# Autodesk Inventor assembly: ASY Вал
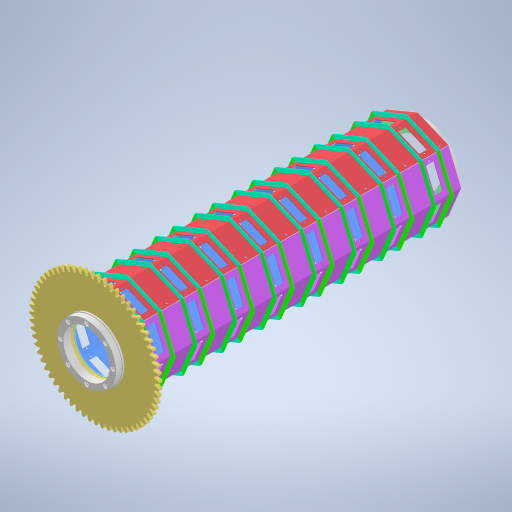
[picture p0: Inventor's stored thumbnail of the model, 512x512]
Saved by Autodesk Inventor 2024.2 (Build 282272000, 272)
## iProperties
Created: 2024-04-28
Part Number: ASY Вал
Document SubType Name: Assembly
Designer: pokla
Author: pokla
## Documents named in this file (13)
- C:\Users\admin\My Drive (bigstupidbeast@gmail.com)\Inventor\Disk Micro filter\ДМФ 06.05.24 21-33\ASY Вал.iam
- C:\Users\admin\My Drive (bigstupidbeast@gmail.com)\Inventor\Disk Micro filter\ДМФ 06.05.24 21-33\ДМС 101 Барабан торец.ipt
- C:\Users\admin\My Drive (bigstupidbeast@gmail.com)\Inventor\Disk Micro filter\ДМФ 06.05.24 21-33\ДМС 100 Барабан Лист №2.ipt
- C:\Users\admin\My Drive (bigstupidbeast@gmail.com)\Inventor\Disk Micro filter\ДМФ 06.05.24 21-33\ДМС 100 Барабан Лист №3.ipt
- C:\Users\admin\My Drive (bigstupidbeast@gmail.com)\Inventor\Disk Micro filter\ДМФ 06.05.24 21-33\ДМС 102 Опорное кольцо вала перед.ipt
- C:\Users\admin\My Drive (bigstupidbeast@gmail.com)\Inventor\Disk Micro filter\ДМФ 06.05.24 21-33\ДМС 103 Полка для крышки.ipt
- C:\Users\admin\My Drive (bigstupidbeast@gmail.com)\Inventor\Disk Micro filter\ДМФ 06.05.24 21-33\ДМС 000 размеры.ipt
- C:\Users\admin\My Drive (bigstupidbeast@gmail.com)\Inventor\Disk Micro filter\ДМФ 06.05.24 21-33\ДМС 105 Шестерня ведомая.ipt
- C:\Users\admin\My Drive (bigstupidbeast@gmail.com)\Inventor\Disk Micro filter\ДМФ 06.05.24 21-33\ДМС 104 Сектор кольца усилителя барабана_CPY.ipt
- C:\Users\admin\My Drive (bigstupidbeast@gmail.com)\Inventor\Disk Micro filter\ДМФ 06.05.24 21-33\ASY ДМФГиД 01010 крышка галка.iam
- C:\Users\admin\My Drive (bigstupidbeast@gmail.com)\Inventor\Disk Micro filter\ДМФ 06.05.24 21-33\ASY ДМФГиД 01011 Кассета.iam
- C:\Users\admin\My Drive (bigstupidbeast@gmail.com)\Inventor\Disk Micro filter\ДМФ 06.05.24 21-33\ДМС 103 Опорное кольцо вала хвост.ipt.ipt
- ДМС 103 Опорное кольцо вала хвост.ipt
## Components (123 placed, 11 different names)
1. ДМС 000 размеры:1
2. ДМС 101 Барабан торец:2 — Rotational:5, Mate:7, Rigid:15, Rigid:16, Mate:8, Flush:1, Flush:2, Mate:9, Flush:3, Flush:4, Mate:10, Flush:5, Flush:6
3. ДМС 101 Барабан торец:1 — Rotational:6
4. ДМС 100 Барабан Лист №2:1 — Rigid:15, Mate:12, Flush:7
5. ДМС 100 Барабан Лист №3:1 — Rigid:16, Mate:11
6. ДМС 102 Опорное кольцо вала перед:1 — Mate:1, Mate:2, Rotational:4, Mate:6, Rotational:5
7. ДМС 103 Полка для крышки:1 — Mate:9, Flush:3, Flush:4
8. ДМС 103 Полка для крышки:2 — Mate:8, Flush:1, Flush:2
9. ДМС 105 Шестерня ведомая:1 — Rotational:4, Mate:6
10. ASY ДМФГиД 01010 крышка галка:1 [sub-assembly] — Mate:10, Flush:5, Flush:6, Rigid:17
11. ДМС 103 Опорное кольцо вала хвост.ipt:1 — Rotational:6
12. ДМС 104 Сектор кольца усилителя барабана_CPY:4 — Rigid:10
13. ДМС 104 Сектор кольца усилителя барабана_CPY:1 — Rigid:8
14. ДМС 104 Сектор кольца усилителя барабана_CPY:5 — Rigid:10, Rigid:11, Rigid:14
15. ДМС 104 Сектор кольца усилителя барабана_CPY:2 — Rigid:8, Rigid:9, Rigid:14
16. ДМС 104 Сектор кольца усилителя барабана_CPY:3 — Rigid:9, Mate:12
17. ДМС 104 Сектор кольца усилителя барабана_CPY:6 — Rigid:11
18. ДМС 104 Сектор кольца усилителя барабана_CPY:7
19. ДМС 104 Сектор кольца усилителя барабана_CPY:8
20. ДМС 104 Сектор кольца усилителя барабана_CPY:21
21. ДМС 104 Сектор кольца усилителя барабана_CPY:28
22. ДМС 104 Сектор кольца усилителя барабана_CPY:35
23. ДМС 104 Сектор кольца усилителя барабана_CPY:42
24. ДМС 104 Сектор кольца усилителя барабана_CPY:9
25. ДМС 104 Сектор кольца усилителя барабана_CPY:10
26. ДМС 104 Сектор кольца усилителя барабана_CPY:22
27. ДМС 104 Сектор кольца усилителя барабана_CPY:29
28. ДМС 104 Сектор кольца усилителя барабана_CPY:36
29. ДМС 104 Сектор кольца усилителя барабана_CPY:43
30. ДМС 104 Сектор кольца усилителя барабана_CPY:11
31. ДМС 104 Сектор кольца усилителя барабана_CPY:12
32. ДМС 104 Сектор кольца усилителя барабана_CPY:23
33. ДМС 104 Сектор кольца усилителя барабана_CPY:30
34. ДМС 104 Сектор кольца усилителя барабана_CPY:37
35. ДМС 104 Сектор кольца усилителя барабана_CPY:44
36. ДМС 104 Сектор кольца усилителя барабана_CPY:13
37. ДМС 104 Сектор кольца усилителя барабана_CPY:14
38. ДМС 104 Сектор кольца усилителя барабана_CPY:24
39. ДМС 104 Сектор кольца усилителя барабана_CPY:31
40. ДМС 104 Сектор кольца усилителя барабана_CPY:38
41. ДМС 104 Сектор кольца усилителя барабана_CPY:45
42. ДМС 104 Сектор кольца усилителя барабана_CPY:15
43. ДМС 104 Сектор кольца усилителя барабана_CPY:16
44. ДМС 104 Сектор кольца усилителя барабана_CPY:25
45. ДМС 104 Сектор кольца усилителя барабана_CPY:32
46. ДМС 104 Сектор кольца усилителя барабана_CPY:39
47. ДМС 104 Сектор кольца усилителя барабана_CPY:46
48. ДМС 104 Сектор кольца усилителя барабана_CPY:17
49. ДМС 104 Сектор кольца усилителя барабана_CPY:18
50. ДМС 104 Сектор кольца усилителя барабана_CPY:26
51. ДМС 104 Сектор кольца усилителя барабана_CPY:33
52. ДМС 104 Сектор кольца усилителя барабана_CPY:40
53. ДМС 104 Сектор кольца усилителя барабана_CPY:47
54. ДМС 104 Сектор кольца усилителя барабана_CPY:19 — Mate:11
55. ДМС 104 Сектор кольца усилителя барабана_CPY:20
56. ДМС 104 Сектор кольца усилителя барабана_CPY:27
57. ДМС 104 Сектор кольца усилителя барабана_CPY:34
58. ДМС 104 Сектор кольца усилителя барабана_CPY:41
59. ДМС 104 Сектор кольца усилителя барабана_CPY:48 — Flush:7
60. ASY ДМФГиД 01011 Кассета:1 [sub-assembly] — Rigid:17
61. ASY ДМФГиД 01011 Кассета:2 [sub-assembly]
62. ASY ДМФГиД 01011 Кассета:3 [sub-assembly]
63. ASY ДМФГиД 01011 Кассета:4 [sub-assembly]
64. ASY ДМФГиД 01011 Кассета:5 [sub-assembly]
65. ASY ДМФГиД 01011 Кассета:6 [sub-assembly]
66. ASY ДМФГиД 01011 Кассета:7 [sub-assembly]
67. ASY ДМФГиД 01011 Кассета:8 [sub-assembly]
68. ASY ДМФГиД 01011 Кассета:9 [sub-assembly]
69. ASY ДМФГиД 01011 Кассета:10 [sub-assembly]
70. ASY ДМФГиД 01011 Кассета:11 [sub-assembly]
71. ASY ДМФГиД 01011 Кассета:12 [sub-assembly]
72. ASY ДМФГиД 01011 Кассета:13 [sub-assembly]
73. ASY ДМФГиД 01011 Кассета:14 [sub-assembly]
74. ASY ДМФГиД 01011 Кассета:15 [sub-assembly]
75. ASY ДМФГиД 01011 Кассета:16 [sub-assembly]
76. ASY ДМФГиД 01011 Кассета:17 [sub-assembly]
77. ASY ДМФГиД 01011 Кассета:18 [sub-assembly]
78. ASY ДМФГиД 01011 Кассета:19 [sub-assembly]
79. ASY ДМФГиД 01011 Кассета:20 [sub-assembly]
80. ASY ДМФГиД 01011 Кассета:21 [sub-assembly]
81. ASY ДМФГиД 01011 Кассета:22 [sub-assembly]
82. ASY ДМФГиД 01011 Кассета:23 [sub-assembly]
83. ASY ДМФГиД 01011 Кассета:24 [sub-assembly]
84. ASY ДМФГиД 01011 Кассета:25 [sub-assembly]
85. ASY ДМФГиД 01011 Кассета:26 [sub-assembly]
86. ASY ДМФГиД 01011 Кассета:27 [sub-assembly]
87. ASY ДМФГиД 01011 Кассета:28 [sub-assembly]
88. ASY ДМФГиД 01011 Кассета:29 [sub-assembly]
89. ASY ДМФГиД 01011 Кассета:30 [sub-assembly]
90. ASY ДМФГиД 01011 Кассета:31 [sub-assembly]
91. ASY ДМФГиД 01011 Кассета:32 [sub-assembly]
92. ASY ДМФГиД 01011 Кассета:33 [sub-assembly]
93. ASY ДМФГиД 01011 Кассета:34 [sub-assembly]
94. ASY ДМФГиД 01011 Кассета:35 [sub-assembly]
95. ASY ДМФГиД 01011 Кассета:36 [sub-assembly]
96. ASY ДМФГиД 01011 Кассета:37 [sub-assembly]
97. ASY ДМФГиД 01011 Кассета:38 [sub-assembly]
98. ASY ДМФГиД 01011 Кассета:39 [sub-assembly]
99. ASY ДМФГиД 01011 Кассета:40 [sub-assembly]
100. ASY ДМФГиД 01011 Кассета:41 [sub-assembly]
101. ASY ДМФГиД 01011 Кассета:42 [sub-assembly]
102. ASY ДМФГиД 01011 Кассета:43 [sub-assembly]
103. ASY ДМФГиД 01011 Кассета:44 [sub-assembly]
104. ASY ДМФГиД 01011 Кассета:45 [sub-assembly]
105. ASY ДМФГиД 01011 Кассета:46 [sub-assembly]
106. ASY ДМФГиД 01011 Кассета:47 [sub-assembly]
107. ASY ДМФГиД 01011 Кассета:48 [sub-assembly]
108. ASY ДМФГиД 01011 Кассета:49 [sub-assembly]
109. ASY ДМФГиД 01011 Кассета:50 [sub-assembly]
110. ASY ДМФГиД 01011 Кассета:51 [sub-assembly]
111. ASY ДМФГиД 01011 Кассета:52 [sub-assembly]
112. ASY ДМФГиД 01011 Кассета:53 [sub-assembly]
113. ASY ДМФГиД 01011 Кассета:54 [sub-assembly]
114. ASY ДМФГиД 01011 Кассета:55 [sub-assembly]
115. ASY ДМФГиД 01011 Кассета:56 [sub-assembly]
116. ASY ДМФГиД 01011 Кассета:57 [sub-assembly]
117. ASY ДМФГиД 01011 Кассета:58 [sub-assembly]
118. ASY ДМФГиД 01011 Кассета:59 [sub-assembly]
119. ASY ДМФГиД 01011 Кассета:60 [sub-assembly]
120. ASY ДМФГиД 01011 Кассета:61 [sub-assembly]
121. ASY ДМФГиД 01011 Кассета:62 [sub-assembly]
122. ASY ДМФГиД 01011 Кассета:63 [sub-assembly]
123. ASY ДМФГиД 01011 Кассета:64 [sub-assembly]
## Component patterns: (8 elements, first: ДМС 104 Сектор кольца усилителя барабана_CPY:4 + ДМС 104 Сектор кольца усилителя барабана_CPY:1 + ДМС 104 Сектор кольца усилителя барабана_CPY:5 + ДМС 104 Сектор кольца усилителя барабана_CPY:2 + ДМС 104 Сектор кольца усилителя барабана_CPY:3 + ДМС 104 Сектор кольца усилителя барабана_CPY:6), (8 elements), (8 elements, first: ASY ДМФГиД 01011 Кассета:1), Component Pattern 13:2 (8 elements), Component Pattern 13:3 (8 elements), Component Pattern 13:4 (8 elements), Component Pattern 13:5 (8 elements), Component Pattern 13:6 (8 elements), Component Pattern 13:7 (8 elements), Component Pattern 13:8 (8 elements)
## Relationships (27: Mate 9, WeldJoint 8, Flush 7, RevoluteJoint 3)
- Rigid:8 [WeldJoint]: ДМС 104 Сектор кольца усилителя барабана_CPY:1 ↔ ДМС 104 Сектор кольца усилителя барабана_CPY:2
- Rigid:9 [WeldJoint]: ДМС 104 Сектор кольца усилителя барабана_CPY:2 ↔ ДМС 104 Сектор кольца усилителя барабана_CPY:3
- Rigid:10 [WeldJoint]: ДМС 104 Сектор кольца усилителя барабана_CPY:4 ↔ ДМС 104 Сектор кольца усилителя барабана_CPY:5
- Rigid:11 [WeldJoint]: ДМС 104 Сектор кольца усилителя барабана_CPY:5 ↔ ДМС 104 Сектор кольца усилителя барабана_CPY:6
- Rigid:14 [WeldJoint] (108 mm): ДМС 104 Сектор кольца усилителя барабана_CPY:5 ↔ ДМС 104 Сектор кольца усилителя барабана_CPY:2
- Mate:1: ДМС 102 Опорное кольцо вала перед:1
- Mate:2: ДМС 102 Опорное кольцо вала перед:1
- Rotational:4 [RevoluteJoint]: ДМС 102 Опорное кольцо вала перед:1 ↔ ДМС 105 Шестерня ведомая:1
- Mate:6: ДМС 102 Опорное кольцо вала перед:1 ↔ ДМС 105 Шестерня ведомая:1
- Rotational:5 [RevoluteJoint] (24 mm): ДМС 101 Барабан торец:2 ↔ ДМС 102 Опорное кольцо вала перед:1
- Mate:7: ДМС 101 Барабан торец:2
- Rigid:15 [WeldJoint]: ДМС 101 Барабан торец:2 ↔ ДМС 100 Барабан Лист №2:1
- Rigid:16 [WeldJoint]: ДМС 101 Барабан торец:2 ↔ ДМС 100 Барабан Лист №3:1
- Mate:8: ДМС 101 Барабан торец:2 ↔ ДМС 103 Полка для крышки:2
- Flush:1 (3 mm): ДМС 101 Барабан торец:2 ↔ ДМС 103 Полка для крышки:2
- Flush:2 (3 mm): ДМС 101 Барабан торец:2 ↔ ДМС 103 Полка для крышки:2
- Mate:9: ДМС 101 Барабан торец:2 ↔ ДМС 103 Полка для крышки:1
- Flush:3 (3 mm): ДМС 101 Барабан торец:2 ↔ ДМС 103 Полка для крышки:1
- Flush:4 (3 mm): ДМС 101 Барабан торец:2 ↔ ДМС 103 Полка для крышки:1
- Mate:10: ДМС 101 Барабан торец:2 ↔ ASY ДМФГиД 01010 крышка галка:1
- Flush:5: ДМС 101 Барабан торец:2 ↔ ASY ДМФГиД 01010 крышка галка:1
- Flush:6: ДМС 101 Барабан торец:2 ↔ ASY ДМФГиД 01010 крышка галка:1
- Mate:11: ДМС 100 Барабан Лист №3:1 ↔ ДМС 104 Сектор кольца усилителя барабана_CPY:19
- Mate:12: ДМС 100 Барабан Лист №2:1 ↔ ДМС 104 Сектор кольца усилителя барабана_CPY:3
- Flush:7 (29 mm): ДМС 100 Барабан Лист №2:1 ↔ ДМС 104 Сектор кольца усилителя барабана_CPY:48
- Rigid:17 [WeldJoint] (5 mm): ASY ДМФГиД 01010 крышка галка:1 ↔ ASY ДМФГиД 01011 Кассета:1
- Rotational:6 [RevoluteJoint]: ДМС 101 Барабан торец:1 ↔ ДМС 103 Опорное кольцо вала хвост.ipt:1
